# Autodesk Inventor assembly: assembly.rev5
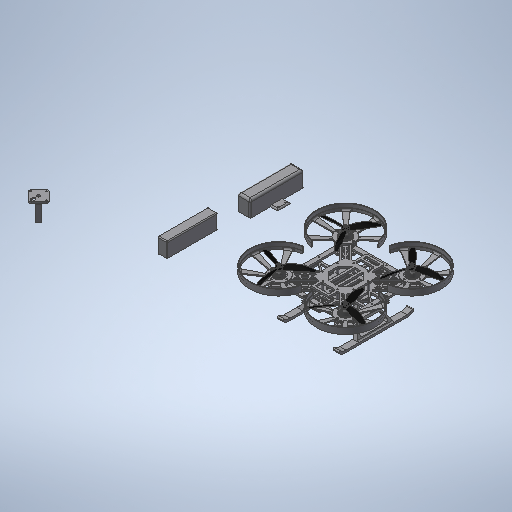
[picture p0: Inventor's stored thumbnail of the model, 512x512]
Saved by Autodesk Inventor 2025.2 (Build 292293000, 293)
## iProperties
Created: 2016-03-08
Part Number: assembly.rev5
Document SubType Name: Assembly
Designer: 200288284
Author: 200288284
## Documents named in this file (11)
- D:\UAV\机架\自制无人机\完整体.iam
- D:\UAV\机架\自制无人机\MOTOR_1806.iam
- D:\UAV\机架\自制无人机\Tri-Blade 5045 Propeller\Tri-Blade 5045 Propeller\5045 CCW.ipt
- D:\UAV\机架\自制无人机\电池.ipt
- D:\UAV\机架\自制无人机\Tri-Blade 5045 Propeller\Protection_for_2.5_inch_prop.ipt
- D:\UAV\机架\自制无人机\底板.ipt
- D:\UAV\机架\自制无人机\中版.ipt
- D:\UAV\机架\自制无人机\顶板.ipt
- D:\UAV\机架\自制无人机\起落架一体.ipt
- D:\UAV\机架\自制无人机\电池仓.ipt
- D:\UAV\机架\自制无人机\新起落架.ipt
## Components (21 placed, 10 different names)
1. 底板:1 — 配合:160, 配合:163, 配合:194, 配合:195, 表面齐平:1, 配合:196, 配合:197, 配合:199, 配合:200, 配合:201
2. 中版:1 — 配合:160, 配合:162, 配合:194, 配合:195, 配合:205
3. 顶板:1 — 配合:162, 配合:163, 配合:178, 配合:179, 配合:180, 配合:181, 配合:182, 配合:184, 配合:185, 配合:187, 配合:192, 配合:193, 配合:202, 配合:203, 配合:205, 配合:206, 配合:207, 配合:208, 配合:209, 配合:210, 配合:211, 配合:213, 配合:214, 配合:215, 配合:216, 配合:222
4. 电池:2 — 配合:192, 配合:222
5. MOTOR_1806:5 [sub-assembly] — 配合:180, 配合:181, 配合:183, 配合:212, 配合:217
6. Protection_for_2.5_inch_prop:5 — 配合:182, 配合:183, 配合:184
7. MOTOR_1806:8 [sub-assembly] — 配合:178, 配合:179, 配合:186, 配合:188, 配合:189, 配合:204
8. Protection_for_2.5_inch_prop:6 — 配合:185, 配合:186, 配合:187
9. 5045 CCW:5 — 配合:188, 配合:189
10. 电池仓:1 — 配合:193
11. 起落架一体:2
12. 新起落架:1 — 表面齐平:1, 配合:196, 配合:197
13. 新起落架:2 — 配合:199, 配合:200, 配合:201
14. Protection_for_2.5_inch_prop:7 — 配合:204, 配合:206, 配合:211
15. Protection_for_2.5_inch_prop:8 — 配合:202, 配合:208, 配合:209
16. Protection_for_2.5_inch_prop:9 — 配合:203, 配合:207, 配合:210
17. 5045 CCW:6 — 配合:218, 配合:220
18. 5045 CCW:7 — 配合:219, 配合:221
19. 5045 CCW:8 — 配合:212, 配合:217
20. MOTOR_1806:9 [sub-assembly] — 配合:213, 配合:216, 配合:218, 配合:220
21. MOTOR_1806:10 [sub-assembly] — 配合:214, 配合:215, 配合:219, 配合:221
## Relationships (46: Mate 45, Flush 1)
- 配合:160 [Mate]: 底板:1 ↔ 中版:1
- 配合:162 [Mate]: 中版:1 ↔ 顶板:1
- 配合:163 [Mate]: 底板:1 ↔ 顶板:1
- 配合:178 [Mate]: 顶板:1 ↔ MOTOR_1806:8
- 配合:179 [Mate]: 顶板:1 ↔ MOTOR_1806:8
- 配合:180 [Mate]: 顶板:1 ↔ MOTOR_1806:5
- 配合:181 [Mate]: 顶板:1 ↔ MOTOR_1806:5
- 配合:182 [Mate]: 顶板:1 ↔ Protection_for_2.5_inch_prop:5
- 配合:183 [Mate]: MOTOR_1806:5 ↔ Protection_for_2.5_inch_prop:5
- 配合:184 [Mate]: 顶板:1 ↔ Protection_for_2.5_inch_prop:5
- 配合:185 [Mate]: 顶板:1 ↔ Protection_for_2.5_inch_prop:6
- 配合:186 [Mate]: MOTOR_1806:8 ↔ Protection_for_2.5_inch_prop:6
- 配合:187 [Mate]: 顶板:1 ↔ Protection_for_2.5_inch_prop:6
- 配合:188 [Mate]: MOTOR_1806:8 ↔ 5045 CCW:5
- 配合:189 [Mate]: MOTOR_1806:8 ↔ 5045 CCW:5
- 配合:192 [Mate]: 顶板:1 ↔ 电池:2
- 配合:193 [Mate]: 顶板:1 ↔ 电池仓:1
- 配合:194 [Mate]: 底板:1 ↔ 中版:1
- 配合:195 [Mate]: 底板:1 ↔ 中版:1
- 表面齐平:1 [Flush]: 底板:1 ↔ 新起落架:1
- 配合:196 [Mate]: 底板:1 ↔ 新起落架:1
- 配合:197 [Mate]: 底板:1 ↔ 新起落架:1
- 配合:199 [Mate]: 底板:1 ↔ 新起落架:2
- 配合:200 [Mate]: 底板:1 ↔ 新起落架:2
- 配合:201 [Mate]: 底板:1 ↔ 新起落架:2
- 配合:202 [Mate]: 顶板:1 ↔ Protection_for_2.5_inch_prop:8
- 配合:203 [Mate]: 顶板:1 ↔ Protection_for_2.5_inch_prop:9
- 配合:204 [Mate]: MOTOR_1806:8 ↔ Protection_for_2.5_inch_prop:7
- 配合:205 [Mate]: 中版:1 ↔ 顶板:1
- 配合:206 [Mate]: 顶板:1 ↔ Protection_for_2.5_inch_prop:7
- 配合:207 [Mate]: 顶板:1 ↔ Protection_for_2.5_inch_prop:9
- 配合:208 [Mate]: 顶板:1 ↔ Protection_for_2.5_inch_prop:8
- 配合:209 [Mate]: 顶板:1 ↔ Protection_for_2.5_inch_prop:8
- 配合:210 [Mate]: 顶板:1 ↔ Protection_for_2.5_inch_prop:9
- 配合:211 [Mate]: 顶板:1 ↔ Protection_for_2.5_inch_prop:7
- 配合:212 [Mate]: MOTOR_1806:5 ↔ 5045 CCW:8
- 配合:213 [Mate]: 顶板:1 ↔ MOTOR_1806:9
- 配合:214 [Mate]: 顶板:1 ↔ MOTOR_1806:10
- 配合:215 [Mate]: 顶板:1 ↔ MOTOR_1806:10
- 配合:216 [Mate]: 顶板:1 ↔ MOTOR_1806:9
- 配合:217 [Mate]: MOTOR_1806:5 ↔ 5045 CCW:8
- 配合:218 [Mate]: 5045 CCW:6 ↔ MOTOR_1806:9
- 配合:219 [Mate]: 5045 CCW:7 ↔ MOTOR_1806:10
- 配合:220 [Mate]: 5045 CCW:6 ↔ MOTOR_1806:9
- 配合:221 [Mate]: 5045 CCW:7 ↔ MOTOR_1806:10
- 配合:222 [Mate]: 顶板:1 ↔ 电池:2
